# Autodesk Inventor assembly: Button Fixture Assembly
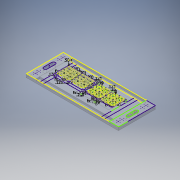
[picture p0: Inventor's stored thumbnail of the model, 180x180]
Saved by Autodesk Inventor 2,016 (Build 200138000, 138)
## iProperties
Created: 2016-07-07
Part Number: Button Fixture Assembly
Document SubType Name: Assembly
Designer: Sam Clay
Author: Sam Clay
## Documents named in this file (3)
- Z:\enclosure\inventor\Button Fixture Assembly.iam
- Z:\enclosure\inventor\Button Fixture Base.ipt
- Z:\enclosure\inventor\Case Buttons CAM.ipt
## Components (17 placed, 2 different names)
1. Button Fixture Base:1 — Planar:4, Mate:5, Mate:6, Mate:7, Mate:8, Mate:9
2. Case Buttons CAM:9
3. Case Buttons CAM:10
4. Case Buttons CAM:11 — Mate:7, Mate:8, Mate:9
5. Case Buttons CAM:12
6. Case Buttons CAM:25
7. Case Buttons CAM:26
8. Case Buttons CAM:27
9. Case Buttons CAM:28
10. Case Buttons CAM:17 — Planar:4, Mate:5, Mate:6
11. Case Buttons CAM:18
12. Case Buttons CAM:19
13. Case Buttons CAM:20
14. Case Buttons CAM:29
15. Case Buttons CAM:30
16. Case Buttons CAM:31
17. Case Buttons CAM:32
## Component patterns: (2 elements), (2 elements), (4 elements, first: Case Buttons CAM:9), Component Pattern 3:2 (4 elements), (4 elements, first: Case Buttons CAM:17), Component Pattern 4:2 (4 elements)
## Relationships (6: Mate 5, PlanarJoint 1)
- Planar:4 (11.43 mm): Button Fixture Base:1 ↔ Case Buttons CAM:17
- Mate:5 (165.1 mm): Button Fixture Base:1 ↔ Case Buttons CAM:17
- Mate:6 (5.08 mm): Button Fixture Base:1 ↔ Case Buttons CAM:17
- Mate:7 (0.7937 mm): Button Fixture Base:1 ↔ Case Buttons CAM:11
- Mate:8 (3.175 mm): Button Fixture Base:1 ↔ Case Buttons CAM:11
- Mate:9 (0.762 mm): Button Fixture Base:1 ↔ Case Buttons CAM:11
